# Autodesk Inventor assembly: 32ch_ECoG_assembled_3p0
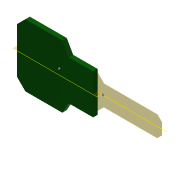
[picture p0: Inventor's stored thumbnail of the model, 180x180]
Saved by Autodesk Inventor 2014 (Build 180170000, 170)
## iProperties
Created: 2016-08-28
Part Number: 32ch_ECoG_assembled_3p0
Document SubType Name: Assembly
Designer: Camilo
Author: Camilo
## Documents named in this file (3)
- Z:\Github\AgingTests\3D parts\ECoG holder_2p0\32ch_ECoG_assembled_3p0.iam
- Z:\Github\AgingTests\3D parts\ECoG holder_2p0\32ch_ACF2TDT_board_3p0.ipt
- Z:\Github\AgingTests\3D parts\ECoG holder_2p0\32ch_ECoG_3p0.ipt
## Components (2 placed, 2 different names)
1. 32ch_ACF2TDT_board_3p0:1 — Flush:2, Flush:1, Mate:1, Mate:4, Mate:3, Mate:2
2. 32ch_ECoG_3p0:1 — Mate:4, Mate:3, Mate:2
## Relationships (6: Mate 4, Flush 2)
- Flush:2: 32ch_ACF2TDT_board_3p0:1
- Flush:1: 32ch_ACF2TDT_board_3p0:1
- Mate:1: 32ch_ACF2TDT_board_3p0:1
- Mate:4 (-7.15 mm): 32ch_ACF2TDT_board_3p0:1 ↔ 32ch_ECoG_3p0:1
- Mate:3: 32ch_ACF2TDT_board_3p0:1 ↔ 32ch_ECoG_3p0:1
- Mate:2: 32ch_ACF2TDT_board_3p0:1 ↔ 32ch_ECoG_3p0:1
